# Autodesk Inventor assembly: Joes_Robot
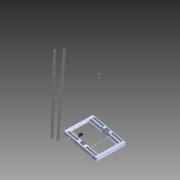
[picture p0: Inventor's stored thumbnail of the model, 180x180]
Saved by Autodesk Inventor 2015 SP1 (Build 190203100, 203)
## iProperties
Created: 2015-01-23
Part Number: Joes_Robot
Document SubType Name: Assembly
Designer: 55221
Author: 55221
## Documents named in this file (15)
- Z:\RoboEaglesCAD\2015CAD\Misc\Joes_Robot.iam
- Z:\RoboEaglesCAD\2015CAD\wheelBase\Outside Sheet Square.ipt
- Z:\RoboEaglesCAD\2015CAD\wheelBase\2x3 Hole Bracket.ipt
- Z:\RoboEaglesCAD\2015CAD\wheelBase\Inside Sheet Square.ipt
- Z:\RoboEaglesCAD\2015CAD\wheelBase\End Sheet Square.ipt
- Z:\RoboEaglesCAD\2015CAD\Motion\GuidanceShaft.ipt
- Z:\RoboEaglesCAD\2015CAD\Motion\Roller.ipt
- Z:\RoboEaglesCAD\2015CAD\wheelBase\churroLong.ipt
- Z:\RoboEaglesCAD\2015CAD\wheelBase\TB Output Shaft Hex L-Base 2.ipt
- Z:\RoboEaglesCAD\2015CAD\wheelBase\GBBearing.ipt
- Z:\RoboEaglesCAD\2015CAD\wheelBase\CIM Motor SW.ipt
- Z:\RoboEaglesCAD\2015CAD\wheelBase\gearBoxSimple\simpleGBHousing.ipt
- Z:\RoboEaglesCAD\2015CAD\wheelBase\gearBoxSimple\simpleGBMount.ipt
- Z:\RoboEaglesCAD\2015CAD\wheelBase\gearBoxSimple\simpleGBStopBlockSmallCylindrical.ipt
- Z:\RoboEaglesCAD\2015CAD\wheelBase\gearBoxSimple\simpleGBStopBlockLargeHex.ipt
## Components (21 placed, 14 different names)
1. Outside Sheet Square:1 — Mate:122, Mate:123, Mate:124, Mate:125, Mate:126, Mate:128, Mate:129
2. 2x3 Hole Bracket:1 — Mate:119, Mate:120, Mate:121, Mate:122, Mate:123
3. 2x3 Hole Bracket:2 — Mate:116, Mate:117, Mate:118, Mate:124
4. Inside Sheet Square:1 — Mate:116, Mate:117, Mate:118, Mate:119, Mate:120, Mate:121, Mate:127, Mate:130, Mate:144
5. End Sheet Square:1 — Mate:125, Mate:126, Mate:127, Mate:139, Mate:140, Mate:141
6. Inside Sheet Square:2 — Mate:131, Mate:132, Mate:134, Mate:136, Mate:137, Mate:141, Mate:143
7. Outside Sheet Square:2 — Mate:133, Mate:135, Mate:138, Mate:139, Mate:140, Mate:142
8. End Sheet Square:2 — Angle:3, Mate:128, Mate:129, Mate:130, Mate:142, Mate:143
9. 2x3 Hole Bracket:3 — Mate:131, Mate:132, Mate:133, Mate:134
10. 2x3 Hole Bracket:4 — Mate:135, Mate:136, Mate:137, Mate:138
11. GuidanceShaft:1
12. GuidanceShaft:2
13. Roller:1
14. churroLong:2
15. GBBearing:2
16. CIM Motor SW:3 — Mate:111, Mate:112
17. simpleGBHousing:1 — Mate:102, Mate:103, Mate:104, Mate:105, Mate:106, Mate:109, Mate:110, Mate:111, Mate:112, Angle:3
18. simpleGBMount:1 — Mate:102, Mate:103, Mate:104
19. TB Output Shaft Hex L-Base 2:3 — Mate:107, Mate:108
20. simpleGBStopBlockSmallCylindrical:1 — Mate:105, Mate:106, Mate:107, Mate:108
21. simpleGBStopBlockLargeHex:1 — Mate:109, Mate:110, Mate:144
## Relationships (41: Mate 40, Angle 1)
- Mate:102: simpleGBHousing:1 ↔ simpleGBMount:1
- Mate:103: simpleGBHousing:1 ↔ simpleGBMount:1
- Mate:104: simpleGBHousing:1 ↔ simpleGBMount:1
- Mate:105: simpleGBHousing:1 ↔ simpleGBStopBlockSmallCylindrical:1
- Mate:106: simpleGBHousing:1 ↔ simpleGBStopBlockSmallCylindrical:1
- Mate:107: TB Output Shaft Hex L-Base 2:3 ↔ simpleGBStopBlockSmallCylindrical:1
- Mate:108: TB Output Shaft Hex L-Base 2:3 ↔ simpleGBStopBlockSmallCylindrical:1
- Mate:109: simpleGBHousing:1 ↔ simpleGBStopBlockLargeHex:1
- Mate:110: simpleGBHousing:1 ↔ simpleGBStopBlockLargeHex:1
- Mate:111: CIM Motor SW:3 ↔ simpleGBHousing:1
- Mate:112: CIM Motor SW:3 ↔ simpleGBHousing:1
- Angle:3 (0 deg): End Sheet Square:2 ↔ simpleGBHousing:1
- Mate:116: 2x3 Hole Bracket:2 ↔ Inside Sheet Square:1
- Mate:117: 2x3 Hole Bracket:2 ↔ Inside Sheet Square:1
- Mate:118: 2x3 Hole Bracket:2 ↔ Inside Sheet Square:1
- Mate:119: 2x3 Hole Bracket:1 ↔ Inside Sheet Square:1
- Mate:120: 2x3 Hole Bracket:1 ↔ Inside Sheet Square:1
- Mate:121: 2x3 Hole Bracket:1 ↔ Inside Sheet Square:1
- Mate:122: Outside Sheet Square:1 ↔ 2x3 Hole Bracket:1
- Mate:123: Outside Sheet Square:1 ↔ 2x3 Hole Bracket:1
- Mate:124: Outside Sheet Square:1 ↔ 2x3 Hole Bracket:2
- Mate:125: Outside Sheet Square:1 ↔ End Sheet Square:1
- Mate:126: Outside Sheet Square:1 ↔ End Sheet Square:1
- Mate:127: Inside Sheet Square:1 ↔ End Sheet Square:1
- Mate:128: Outside Sheet Square:1 ↔ End Sheet Square:2
- Mate:129: Outside Sheet Square:1 ↔ End Sheet Square:2
- Mate:130: Inside Sheet Square:1 ↔ End Sheet Square:2
- Mate:131: Inside Sheet Square:2 ↔ 2x3 Hole Bracket:3
- Mate:132: Inside Sheet Square:2 ↔ 2x3 Hole Bracket:3
- Mate:133: Outside Sheet Square:2 ↔ 2x3 Hole Bracket:3
- Mate:134: Inside Sheet Square:2 ↔ 2x3 Hole Bracket:3
- Mate:135: Outside Sheet Square:2 ↔ 2x3 Hole Bracket:4
- Mate:136: Inside Sheet Square:2 ↔ 2x3 Hole Bracket:4
- Mate:137: Inside Sheet Square:2 ↔ 2x3 Hole Bracket:4
- Mate:138: Outside Sheet Square:2 ↔ 2x3 Hole Bracket:4
- Mate:139: End Sheet Square:1 ↔ Outside Sheet Square:2
- Mate:140: End Sheet Square:1 ↔ Outside Sheet Square:2
- Mate:141: End Sheet Square:1 ↔ Inside Sheet Square:2
- Mate:142: Outside Sheet Square:2 ↔ End Sheet Square:2
- Mate:143: Inside Sheet Square:2 ↔ End Sheet Square:2
- Mate:144: Inside Sheet Square:1 ↔ simpleGBStopBlockLargeHex:1
